# Autodesk Inventor assembly: Sprzęgło
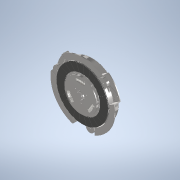
[picture p0: Inventor's stored thumbnail of the model, 180x180]
Saved by Autodesk Inventor 2022 (Build 260153000, 153)
## iProperties
Created: 2021-11-28
Part Number: Sprzęgło
Document SubType Name: Assembly
Designer: Mateu
Author: Mateu
## Documents named in this file (7)
- C:\Users\Mateu\Documents\GitHub\ToyotaStarletClutch\Clutch.iam
- C:\Users\Mateu\Documents\GitHub\ToyotaStarletClutch\ClutchDrivePlate.iam
- C:\Users\Mateu\Documents\GitHub\ToyotaStarletClutch\Clutch_Shaft.ipt
- C:\Users\Mateu\Documents\GitHub\ToyotaStarletClutch\ClutchPressurePlate.iam
- C:\Users\Mateu\Documents\GitHub\ToyotaStarletClutch\Clutch_Bearing.iam
- C:\Users\Mateu\Documents\GitHub\ToyotaStarletClutch\Clutch_BearingCover.ipt
- C:\Users\Mateu\Documents\GitHub\ToyotaStarletClutch\OldVersions\dsyknekwx.fres
## Components (5 placed, 5 different names)
1. ClutchDrivePlate:1 [sub-assembly] — Wstawiające:1, Wstawiające:2
2. Clutch_Shaft:1 — Wstawiające:1, Wstawiające:3, Równoległe:1
3. ClutchPressurePlate:1 [sub-assembly] — Wstawiające:2
4. Clutch_Bearing [sub-assembly] — Wstawiające:3, Równoległe:2
5. Clutch_BearingCover:1 — Równoległe:1, Równoległe:2
## Relationships (5: Insert 3, Flush 2)
- Wstawiające:1 [Insert] (-20 mm): ClutchDrivePlate:1 ↔ Clutch_Shaft:1
- Wstawiające:2 [Insert] (1 mm): ClutchDrivePlate:1 ↔ ClutchPressurePlate:1
- Wstawiające:3 [Insert] (-25 mm): Clutch_Shaft:1 ↔ Clutch_Bearing
- Równoległe:1 [Flush]: Clutch_Shaft:1 ↔ Clutch_BearingCover:1
- Równoległe:2 [Flush]: Clutch_Bearing ↔ Clutch_BearingCover:1
